# Autodesk Inventor assembly: knoppendoosje
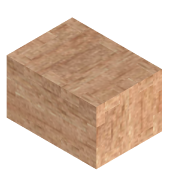
[picture p0: Inventor's stored thumbnail of the model, 180x180]
Saved by Autodesk Inventor 2020.3 (Build 243373000, 373)
## iProperties
Created: 2020-12-08
Part Number: knoppendoosje
Document SubType Name: Assembly
Designer: Svend
Author: Svend
## Documents named in this file (7)
- C:\Users\Svend\OneDrive\Documents\GitHub\Rolstoel\knoppendoosje.iam
- C:\Users\Svend\OneDrive\Documents\GitHub\Rolstoel\knop op en neer.ipt
- C:\Users\Svend\OneDrive\Documents\GitHub\Rolstoel\voorkant knoppendoosje.ipt
- C:\Users\Svend\OneDrive\Documents\GitHub\Rolstoel\zijkant knoppendoosje.ipt
- C:\Users\Svend\OneDrive\Documents\GitHub\Rolstoel\achterkant knoppendoosje.ipt
- C:\Users\Svend\OneDrive\Documents\GitHub\Rolstoel\onderkantBovenkant knoppendoosje.ipt
- C:\Users\Svend\OneDrive\Documents\GitHub\Rolstoel\zijkant knoppendoosje met gat.ipt
## Components (8 placed, 6 different names)
1. knop op en neer:1 — Flush:1, Mate:2, Mate:3, Mate:4, Mate:6
2. knop op en neer:2 — Flush:1, Mate:2, Mate:3, Mate:5
3. voorkant knoppendoosje:1 — Mate:4, Mate:5, Mate:6, Flush:2, Flush:3, Mate:7, Flush:4, Flush:5, Flush:6, Flush:7, Mate:8, Flush:15
4. zijkant knoppendoosje:1 — Flush:2, Flush:3, Flush:6, Flush:7, Flush:8, Flush:9, Flush:10, Flush:12, Flush:14, Flush:16
5. zijkant knoppendoosje met gat:2 — Mate:7, Flush:4, Flush:5, Flush:11
6. achterkant knoppendoosje:1 — Flush:8, Flush:9, Flush:10, Flush:13
7. onderkantBovenkant knoppendoosje:1 — Flush:11, Flush:12, Flush:13, Flush:14
8. onderkantBovenkant knoppendoosje:2 — Mate:8, Flush:15, Flush:16
## Relationships (23: Flush 16, Mate 7)
- Flush:1: knop op en neer:1 ↔ knop op en neer:2
- Mate:2 (25 mm): knop op en neer:1 ↔ knop op en neer:2
- Mate:3: knop op en neer:1 ↔ knop op en neer:2
- Mate:4: knop op en neer:1 ↔ voorkant knoppendoosje:1
- Mate:5: knop op en neer:2 ↔ voorkant knoppendoosje:1
- Mate:6: knop op en neer:1 ↔ voorkant knoppendoosje:1
- Flush:2: voorkant knoppendoosje:1 ↔ zijkant knoppendoosje:1
- Flush:3: voorkant knoppendoosje:1 ↔ zijkant knoppendoosje:1
- Mate:7: voorkant knoppendoosje:1 ↔ zijkant knoppendoosje met gat:2
- Flush:4: voorkant knoppendoosje:1 ↔ zijkant knoppendoosje met gat:2
- Flush:5: voorkant knoppendoosje:1 ↔ zijkant knoppendoosje met gat:2
- Flush:6: voorkant knoppendoosje:1 ↔ zijkant knoppendoosje:1
- Flush:7: voorkant knoppendoosje:1 ↔ zijkant knoppendoosje:1
- Flush:8: zijkant knoppendoosje:1 ↔ achterkant knoppendoosje:1
- Flush:9: zijkant knoppendoosje:1 ↔ achterkant knoppendoosje:1
- Flush:10: zijkant knoppendoosje:1 ↔ achterkant knoppendoosje:1
- Flush:11: zijkant knoppendoosje met gat:2 ↔ onderkantBovenkant knoppendoosje:1
- Flush:12: zijkant knoppendoosje:1 ↔ onderkantBovenkant knoppendoosje:1
- Flush:13: achterkant knoppendoosje:1 ↔ onderkantBovenkant knoppendoosje:1
- Flush:14: zijkant knoppendoosje:1 ↔ onderkantBovenkant knoppendoosje:1
- Mate:8: voorkant knoppendoosje:1 ↔ onderkantBovenkant knoppendoosje:2
- Flush:15: voorkant knoppendoosje:1 ↔ onderkantBovenkant knoppendoosje:2
- Flush:16: zijkant knoppendoosje:1 ↔ onderkantBovenkant knoppendoosje:2
